# Autodesk Inventor assembly: WormAssy
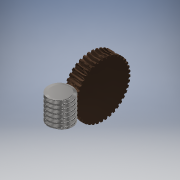
[picture p0: Inventor's stored thumbnail of the model, 180x180]
Saved by Autodesk Inventor 2019.4 (Build 234330000, 330)
## iProperties
Created: 2021-11-21
Part Number: WormAssy
Document SubType Name: Assembly
Designer: Ilija Jovanovic
Author: Ilija Jovanovic
## Documents named in this file (3)
- D:\Git\ParametricWormGear\WormAssy.iam
- D:\Git\ParametricWormGear\Worm.ipt
- D:\Git\ParametricWormGear\WormWheel.ipt
## Components (2 placed, 2 different names)
1. Worm:1 — Mate:1, Mate:2
2. WormWheel:1 — Mate:3, Mate:4, Mate:5
## Relationships (5: Mate 5)
- Mate:1: Worm:1
- Mate:2 (-15 mm): Worm:1
- Mate:3 (-7.5 mm): WormWheel:1
- Mate:4 (42.5 mm): WormWheel:1
- Mate:5 (-0.241 mm): WormWheel:1
## Named parameters: PitchDiam = 25 mm, FaceWidth = 30 mm, PitchDiamWheel = 60 mm, FaceWidthWheel = 15 mm
